# Autodesk Inventor assembly: NEMA17 pancake motor (23mm)
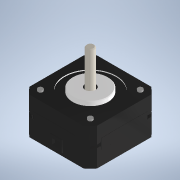
[picture p0: Inventor's stored thumbnail of the model, 180x180]
Saved by Autodesk Inventor 2020 (Build 240168000, 168)
## iProperties
Created: 2021-03-28
Part Number: NEMA17 pancake motor (23mm)
Document SubType Name: Assembly
Designer: AOB
Mass: 198.343 g
Surface Area: 226.811 cm^2
Volume: 25.2667 cm^3
Density: 7.85 g/cm^3
Author: AOB
## Documents named in this file (3)
- C:\Users\marti\Documents\Inventor\ProjectBoron\Boron Ultima\NEMA17 pancake motor (23mm).iam
- C:\Users\marti\Documents\Inventor\ProjectBoron\Boron Ultima\nema17 pancake bottom.ipt
- C:\Users\marti\Documents\Inventor\ProjectBoron\Boron Ultima\NEMA17 pancake top.ipt
## Components (2 placed, 2 different names)
1. nema17 pancake bottom:1 — Flush:1, Flush:2, Mate:1
2. NEMA17 pancake top:1 — Flush:1, Flush:2, Mate:1
## Relationships (3: Flush 2, Mate 1)
- Flush:1: nema17 pancake bottom:1 ↔ NEMA17 pancake top:1
- Flush:2: nema17 pancake bottom:1 ↔ NEMA17 pancake top:1
- Mate:1: nema17 pancake bottom:1 ↔ NEMA17 pancake top:1
